# Autodesk Inventor assembly: ASY МОО 020 конус
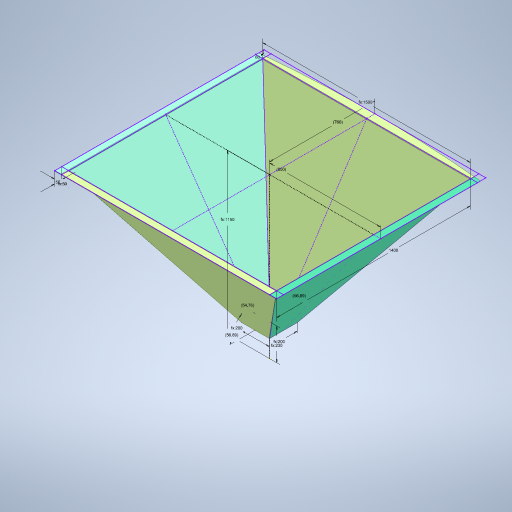
[picture p0: Inventor's stored thumbnail of the model, 512x512]
Saved by Autodesk Inventor 2024.2 (Build 282272000, 272)
## iProperties
Created: 2024-05-19
Part Number: ASY МОО 020 конус
Document SubType Name: Assembly
Designer: admin
Author: admin
## Documents named in this file (7)
- C:\Users\pokla\Documents\Inventor\Manturovo_Se-clar-Gleb\ASY МОО 020 конус.iam
- C:\Users\pokla\Documents\Inventor\Manturovo_Se-clar-Gleb\конус\МОО 023 конус правый борт 1.ipt
- C:\Users\pokla\Documents\Inventor\Manturovo_Se-clar-Gleb\конус\МОО 029 конус дно.ipt
- C:\Users\pokla\Documents\Inventor\Manturovo_Se-clar-Gleb\конус\МОО 025 конус левый борт 1.ipt
- C:\Users\pokla\Documents\Inventor\Manturovo_Se-clar-Gleb\конус\МОО 022 конус корма.ipt
- C:\Users\pokla\Documents\Inventor\Manturovo_Se-clar-Gleb\конус\МОО 021 конус эскиз .ipt
- C:\Users\pokla\Documents\Inventor\Manturovo_Se-clar-Gleb\конус\МОО 026 конус нос.ipt
## Components (6 placed, 6 different names)
1. МОО 021 конус эскиз :1 — Flush:8, Flush:9, Mate:1
2. МОО 022 конус корма:1 — Flush:6, Flush:10, Mate:2
3. МОО 029 конус дно:1 — Flush:4, Flush:5, Flush:11
4. МОО 023 конус правый борт 1:1 — Flush:13, Flush:14, Flush:15
5. МОО 025 конус левый борт 1:1 — Mate:3, Flush:12, Mate:4
6. МОО 026 конус нос:1 — Flush:16, Mate:5, Flush:17
## Relationships (18: Flush 13, Mate 5)
- Flush:4: МОО 029 конус дно:1
- Flush:5: МОО 029 конус дно:1
- Flush:6: МОО 022 конус корма:1
- Flush:8: МОО 021 конус эскиз :1
- Flush:9: МОО 021 конус эскиз :1
- Mate:1: МОО 021 конус эскиз :1
- Flush:10: МОО 022 конус корма:1
- Mate:2: МОО 022 конус корма:1
- Flush:11 (-230 mm): МОО 029 конус дно:1
- Mate:3: МОО 025 конус левый борт 1:1
- Flush:12: МОО 025 конус левый борт 1:1
- Mate:4: МОО 025 конус левый борт 1:1
- Flush:13: МОО 023 конус правый борт 1:1
- Flush:14: МОО 023 конус правый борт 1:1
- Flush:15: МОО 023 конус правый борт 1:1
- Flush:16: МОО 026 конус нос:1
- Mate:5: МОО 026 конус нос:1
- Flush:17: МОО 026 конус нос:1
